# Autodesk Inventor assembly: Assembly1
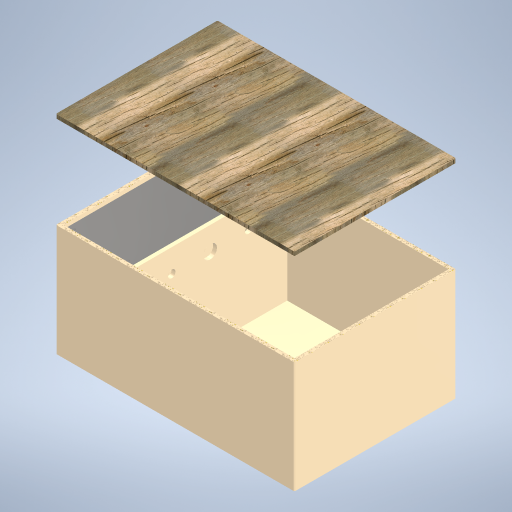
[picture p0: Inventor's stored thumbnail of the model, 512x512]
Saved by Autodesk Inventor 2023.1 (Build 271208000, 208)
## iProperties
Created: 2024-03-27
Part Number: Assembly1
Document SubType Name: Assembly
Designer: bahariridwan
Author: bahariridwan
## Documents named in this file (4)
- C:\Users\bahariridwan\Documents\Design3D\Box_Deteksi_Pembusukan\Assembly1.iam
- C:\Users\bahariridwan\Documents\Design3D\Box_Deteksi_Pembusukan\Box.ipt
- C:\Users\bahariridwan\Documents\Design3D\Box_Deteksi_Pembusukan\Tutup_Box.ipt
- C:\Users\bahariridwan\Documents\Design3D\Box_Deteksi_Pembusukan\Tutup_system.ipt
## Components (3 placed, 3 different names)
1. Box:1 — Mate:1, Mate:2, Flush:1, Flush:2, Flush:3, Flush:4
2. Tutup_Box:1 — Flush:3, Flush:4
3. Tutup_system:1 — Mate:1, Mate:2, Flush:1, Flush:2
## Relationships (6: Flush 4, Mate 2)
- Mate:1: Box:1 ↔ Tutup_system:1
- Mate:2: Box:1 ↔ Tutup_system:1
- Flush:1: Box:1 ↔ Tutup_system:1
- Flush:2: Box:1 ↔ Tutup_system:1
- Flush:3: Box:1 ↔ Tutup_Box:1
- Flush:4: Box:1 ↔ Tutup_Box:1
